# Autodesk Inventor assembly: Ensamble caja de paracaidas
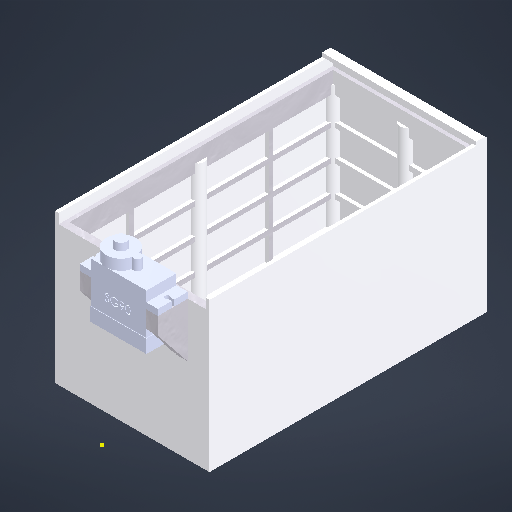
[picture p0: Inventor's stored thumbnail of the model, 512x512]
Saved by Autodesk Inventor 2026 (Build 300175000, 175)
## iProperties
Created: 2026-02-27
Part Number: Ensamble caja de paracaidas
Document SubType Name: Assembly
Designer: Usuario2
Author: Usuario2
## Documents named in this file (3)
- C:\Users\Usuario2\Downloads\Nueva carpeta\Ensamble caja de paracaidas.iam
- C:\Users\Usuario2\Downloads\Nueva carpeta\sg90 micro servo.ipt
- C:\Users\Usuario2\Downloads\Nueva carpeta\Caja sin ranura sin huecos.ipt
## Components (2 placed, 2 different names)
1. sg90 micro servo:1 — Mate:1, Mate:2, Flush:1
2. Caja sin ranura sin huecos:1 — Mate:1, Mate:2, Flush:1
## Relationships (3: Mate 2, Flush 1)
- Mate:1: sg90 micro servo:1 ↔ Caja sin ranura sin huecos:1
- Mate:2: sg90 micro servo:1 ↔ Caja sin ranura sin huecos:1
- Flush:1: sg90 micro servo:1 ↔ Caja sin ranura sin huecos:1
